# Autodesk Inventor assembly: Cooper
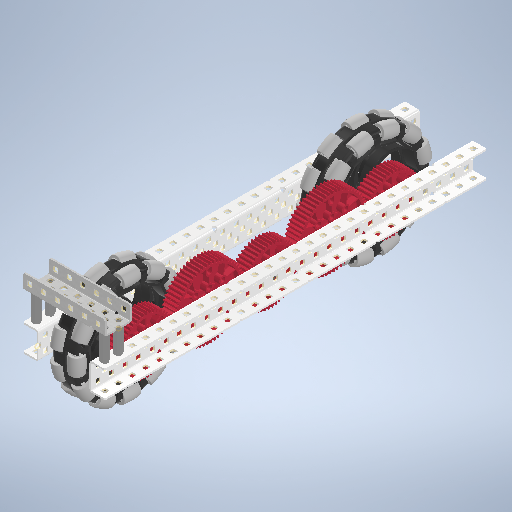
[picture p0: Inventor's stored thumbnail of the model, 512x512]
Saved by Autodesk Inventor 2025.1 (Build 291241000, 241)
## iProperties
Created: 2024-09-09
Part Number: Cooper
Document SubType Name: Assembly
Designer: cssto
Author: cssto
## Documents named in this file (10)
- C:\Users\cssto\OneDrive\Documents\GitHub\ATUM-V5RC-High-Stakes-CAD\Protobot\Cooper.iam
- C:\Users\cssto\OneDrive\Documents\GitHub\ATUM-V5RC-High-Stakes-CAD\VEX-CAD-Inventor\Structure\C Channel\Aluminum 1x2x1\Alu C 1x2x1x28.ipt
- C:\Users\cssto\OneDrive\Documents\GitHub\ATUM-V5RC-High-Stakes-CAD\VEX-CAD-Inventor\Structure\C Channel\Aluminum 1x2x1\Alu C 1x2x1x6.ipt
- C:\Users\cssto\OneDrive\Documents\GitHub\ATUM-V5RC-High-Stakes-CAD\VEX-CAD-Inventor\Structure\Standoff\Standoff 1.00.ipt
- C:\Users\cssto\OneDrive\Documents\GitHub\ATUM-V5RC-High-Stakes-CAD\VEX-CAD-Inventor\Structure\Standoff.ipt
- C:\Users\cssto\OneDrive\Documents\GitHub\ATUM-V5RC-High-Stakes-CAD\VEX-CAD-Inventor\Motion\Gears\HS Gear\HS 60T Gear, Square.iam
- C:\Users\cssto\OneDrive\Documents\GitHub\ATUM-V5RC-High-Stakes-CAD\VEX-CAD-Inventor\Motion\Gears\HS Gear.iam
- C:\Users\cssto\OneDrive\Documents\GitHub\ATUM-V5RC-High-Stakes-CAD\VEX-CAD-Inventor\Motion\Gears\HS Gear\HS 48T Gear, Circle.iam
- C:\Users\cssto\OneDrive\Documents\GitHub\ATUM-V5RC-High-Stakes-CAD\VEX-CAD-Inventor\Motion\Wheels\Omni Wheel\4 Omni, Circle.iam
- C:\Users\cssto\OneDrive\Documents\GitHub\ATUM-V5RC-High-Stakes-CAD\VEX-CAD-Inventor\Motion\Wheels\Omni Wheel.iam
## Components (14 placed, 6 different names)
1. Alu C 1x2x1x28:1 — Rigid:3, Rigid:4, Rotational:4
2. Alu C 1x2x1x28:2 — Rigid:5, Rigid:6, Rotational:5, Rotational:6, Rotational:7, Rotational:8
3. Alu C 1x2x1x6:1 — Rigid:7, Rotational:1, Rotational:2
4. Standoff 1.00:1 — Rigid:3, Rotational:1
5. Standoff 1.00:2 — Rigid:4, Rotational:2
6. Standoff 1.00:3 — Rigid:5
7. Standoff 1.00:4 — Rigid:6, Rigid:7
8. HS 60T Gear, Square:2 [sub-assembly] — Rotational:7
9. HS 60T Gear, Square:3 [sub-assembly] — Rotational:5
10. HS 48T Gear, Circle:5 [sub-assembly] — Rotational:3
11. HS 48T Gear, Circle:7 [sub-assembly] — Rotational:6
12. HS 48T Gear, Circle:8 [sub-assembly] — Rigid:8, Rotational:8
13. 4 Omni, Circle:1 [sub-assembly] — Rigid:8
14. 4 Omni, Circle:2 [sub-assembly] — Rotational:3, Rotational:4
## Relationships (14: RevoluteJoint 8, WeldJoint 6)
- Rigid:3 [WeldJoint]: Alu C 1x2x1x28:1 ↔ Standoff 1.00:1
- Rigid:4 [WeldJoint]: Alu C 1x2x1x28:1 ↔ Standoff 1.00:2
- Rigid:5 [WeldJoint]: Alu C 1x2x1x28:2 ↔ Standoff 1.00:3
- Rigid:6 [WeldJoint]: Alu C 1x2x1x28:2 ↔ Standoff 1.00:4
- Rigid:7 [WeldJoint]: Alu C 1x2x1x6:1 ↔ Standoff 1.00:4
- Rotational:1 [RevoluteJoint]: Alu C 1x2x1x6:1 ↔ Standoff 1.00:1
- Rotational:2 [RevoluteJoint]: Alu C 1x2x1x6:1 ↔ Standoff 1.00:2
- Rotational:3 [RevoluteJoint] (5.08 mm): HS 48T Gear, Circle:5 ↔ 4 Omni, Circle:2
- Rotational:4 [RevoluteJoint] (8.89 mm): Alu C 1x2x1x28:1 ↔ 4 Omni, Circle:2
- Rigid:8 [WeldJoint] (-5.08 mm): HS 48T Gear, Circle:8 ↔ 4 Omni, Circle:1
- Rotational:5 [RevoluteJoint] (2.54 mm): Alu C 1x2x1x28:2 ↔ HS 60T Gear, Square:3
- Rotational:6 [RevoluteJoint] (2.54 mm): Alu C 1x2x1x28:2 ↔ HS 48T Gear, Circle:7
- Rotational:7 [RevoluteJoint] (2.54 mm): Alu C 1x2x1x28:2 ↔ HS 60T Gear, Square:2
- Rotational:8 [RevoluteJoint] (3.81 mm): Alu C 1x2x1x28:2 ↔ HS 48T Gear, Circle:8
